# Autodesk Inventor assembly: Baugruppe Test 1
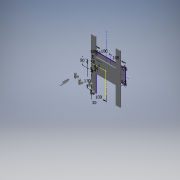
[picture p0: Inventor's stored thumbnail of the model, 180x180]
Saved by Autodesk Inventor 2018 (Build 220112000, 112)
## iProperties
Created: 2018-01-20
Part Number: Baugruppe Test 1
Material: Generisch
Document SubType Name: Assembly
Designer: Administrator
Author: Administrator
## Documents named in this file (6)
- C:\Users\Administrator\Desktop\Baugruppe Test 1.iam
- C:\Users\Administrator\Desktop\Achsenhalterung.ipt
- C:\Users\Administrator\Desktop\Platzhalter Zylinder Groß.ipt
- C:\Users\Administrator\Desktop\Platzhalter Zylinder Klein.ipt
- C:\Users\Administrator\Desktop\Chassis-2.ipt
- C:\Users\Administrator\Desktop\Chassis-1.ipt
## Components (14 placed, 5 different names)
1. Achsenhalterung:1
2. Achsenhalterung:2
3. Achsenhalterung:3
4. Achsenhalterung:4
5. Platzhalter Zylinder Groß:1
6. Platzhalter Zylinder Groß:2
7. Platzhalter Zylinder Groß:3
8. Platzhalter Zylinder Groß:4
9. Platzhalter Zylinder Klein:1 — Starr:4, Starr:5
10. Platzhalter Zylinder Klein:2 — Starr:2
11. Platzhalter Zylinder Klein:3 — Starr:6
12. Platzhalter Zylinder Klein:4 — Starr:1
13. Chassis-2:1 — Starr:5, Starr:6
14. Chassis-1:1 — Starr:2, Starr:4, Starr:1
## Relationships (5: WeldJoint 5)
- Starr:2 [WeldJoint]: Platzhalter Zylinder Klein:2 ↔ Chassis-1:1
- Starr:4 [WeldJoint]: Platzhalter Zylinder Klein:1 ↔ Chassis-1:1
- Starr:1 [WeldJoint]: Platzhalter Zylinder Klein:4 ↔ Chassis-1:1
- Starr:5 [WeldJoint]: Platzhalter Zylinder Klein:1 ↔ Chassis-2:1
- Starr:6 [WeldJoint]: Platzhalter Zylinder Klein:3 ↔ Chassis-2:1
